# Autodesk Inventor assembly: Full
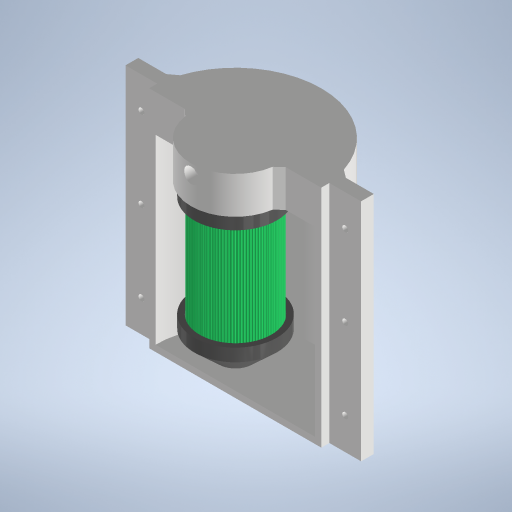
[picture p0: Inventor's stored thumbnail of the model, 512x512]
Saved by Autodesk Inventor 2024 (Build 280153020, 153B)
## iProperties
Created: 2023-07-10
Part Number: Full
Document SubType Name: Assembly
Designer: torban
Author: torban
## Documents named in this file (3)
- D:\GIT\CIRC-2023-Night-Task-HW-SW\CAD\Reactor\Reactor\Full.iam
- D:\GIT\CIRC-2023-Night-Task-HW-SW\CAD\Reactor Module\Reactor Module\Final.iam
- D:\GIT\CIRC-2023-Night-Task-HW-SW\CAD\Reactor\Reactor\Reactor Receptacle.ipt
## Components (2 placed, 2 different names)
1. Final:1 [sub-assembly] — Mate:1, Mate:2
2. Reactor Receptacle:1 — Mate:1, Mate:2
## Relationships (2: Mate 2)
- Mate:1: Final:1 ↔ Reactor Receptacle:1
- Mate:2: Final:1 ↔ Reactor Receptacle:1
